# Autodesk Inventor assembly: Hexapod
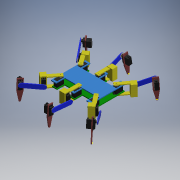
[picture p0: Inventor's stored thumbnail of the model, 180x180]
Saved by Autodesk Inventor 2017 (Build 210142000, 142)
## iProperties
Part Number: Hexapod
Document SubType Name: Assembly
Designer: alex-
Author: alex-
## Documents named in this file (7)
- D:\Alexander Miller\Documents\Git\Hexapod\3DParts\Hexapod.iam
- D:\Alexander Miller\Documents\Git\Hexapod\3DParts\Body_bottom.ipt
- D:\Alexander Miller\Documents\Git\Hexapod\3DParts\Serov_with_arm.iam
- D:\Alexander Miller\Documents\Git\Hexapod\3DParts\Body_top.ipt
- D:\Alexander Miller\Documents\Git\Hexapod\3DParts\Upper_leg.ipt
- D:\Alexander Miller\Documents\Git\Hexapod\3DParts\Middle_leg.ipt
- D:\Alexander Miller\Documents\Git\Hexapod\3DParts\Lower_leg.ipt
## Components (38 placed, 6 different names)
1. Body_bottom:1 — Rigid:1, Rigid:2, Rigid:3, Rigid:4, Rigid:5, Rigid:6
2. Serov_with_arm:1 [sub-assembly] — Rigid:1, Rigid:7, Rigid:40
3. Serov_with_arm:2 [sub-assembly] — Rigid:2, Rigid:41
4. Serov_with_arm:3 [sub-assembly] — Rigid:4, Rigid:42
5. Serov_with_arm:4 [sub-assembly] — Rigid:6, Rigid:43
6. Serov_with_arm:5 [sub-assembly] — Rigid:3, Rigid:39
7. Serov_with_arm:6 [sub-assembly] — Rigid:5, Rigid:38
8. Body_top:1 — Rigid:7
9. Upper_leg:1 — Rigid:8, Rigid:38
10. Upper_leg:2 — Rigid:15, Rigid:39
11. Upper_leg:3 — Rigid:16, Rigid:40
12. Upper_leg:4 — Rigid:19, Rigid:41
13. Upper_leg:5 — Rigid:18, Rigid:42
14. Upper_leg:6 — Rigid:17, Rigid:43
15. Serov_with_arm:7 [sub-assembly] — Rigid:8, Rigid:20
16. Serov_with_arm:8 [sub-assembly] — Rigid:17, Rigid:22
17. Serov_with_arm:9 [sub-assembly] — Rigid:19, Rigid:25
18. Serov_with_arm:10 [sub-assembly] — Rigid:16, Rigid:23
19. Serov_with_arm:11 [sub-assembly] — Rigid:18, Rigid:24
20. Serov_with_arm:12 [sub-assembly] — Rigid:15, Rigid:21
21. Middle_leg:1 — Rigid:20, Rigid:27
22. Middle_leg:2 — Rigid:22, Rigid:35
23. Middle_leg:3 — Rigid:25, Rigid:37
24. Middle_leg:4 — Rigid:24, Rigid:36
25. Middle_leg:5 — Rigid:23, Rigid:33
26. Middle_leg:6 — Rigid:21, Rigid:34
27. Serov_with_arm:13 [sub-assembly] — Rigid:26, Rigid:27
28. Serov_with_arm:14 [sub-assembly] — Rigid:28, Rigid:36
29. Serov_with_arm:15 [sub-assembly] — Rigid:30, Rigid:37
30. Serov_with_arm:16 [sub-assembly] — Rigid:32, Rigid:34
31. Serov_with_arm:17 [sub-assembly] — Rigid:31, Rigid:35
32. Serov_with_arm:18 [sub-assembly] — Rigid:29, Rigid:33
33. Lower_leg:1 — Rigid:26
34. Lower_leg:2 — Rigid:28
35. Lower_leg:3 — Rigid:29
36. Lower_leg:4 — Rigid:30
37. Lower_leg:5 — Rigid:31
38. Lower_leg:6 — Rigid:32
## Relationships (37: WeldJoint 37)
- Rigid:1 [WeldJoint]: Body_bottom:1 ↔ Serov_with_arm:1
- Rigid:2 [WeldJoint]: Body_bottom:1 ↔ Serov_with_arm:2
- Rigid:3 [WeldJoint]: Body_bottom:1 ↔ Serov_with_arm:5
- Rigid:4 [WeldJoint]: Body_bottom:1 ↔ Serov_with_arm:3
- Rigid:5 [WeldJoint]: Body_bottom:1 ↔ Serov_with_arm:6
- Rigid:6 [WeldJoint]: Body_bottom:1 ↔ Serov_with_arm:4
- Rigid:7 [WeldJoint]: Serov_with_arm:1 ↔ Body_top:1
- Rigid:8 [WeldJoint]: Upper_leg:1 ↔ Serov_with_arm:7
- Rigid:15 [WeldJoint]: Upper_leg:2 ↔ Serov_with_arm:12
- Rigid:16 [WeldJoint]: Upper_leg:3 ↔ Serov_with_arm:10
- Rigid:17 [WeldJoint]: Upper_leg:6 ↔ Serov_with_arm:8
- Rigid:18 [WeldJoint]: Upper_leg:5 ↔ Serov_with_arm:11
- Rigid:19 [WeldJoint]: Upper_leg:4 ↔ Serov_with_arm:9
- Rigid:20 [WeldJoint]: Serov_with_arm:7 ↔ Middle_leg:1
- Rigid:21 [WeldJoint]: Serov_with_arm:12 ↔ Middle_leg:6
- Rigid:23 [WeldJoint]: Serov_with_arm:10 ↔ Middle_leg:5
- Rigid:22 [WeldJoint]: Serov_with_arm:8 ↔ Middle_leg:2
- Rigid:24 [WeldJoint]: Serov_with_arm:11 ↔ Middle_leg:4
- Rigid:25 [WeldJoint]: Serov_with_arm:9 ↔ Middle_leg:3
- Rigid:26 [WeldJoint]: Serov_with_arm:13 ↔ Lower_leg:1
- Rigid:27 [WeldJoint]: Middle_leg:1 ↔ Serov_with_arm:13
- Rigid:28 [WeldJoint]: Serov_with_arm:14 ↔ Lower_leg:2
- Rigid:29 [WeldJoint]: Serov_with_arm:18 ↔ Lower_leg:3
- Rigid:30 [WeldJoint]: Serov_with_arm:15 ↔ Lower_leg:4
- Rigid:31 [WeldJoint]: Serov_with_arm:17 ↔ Lower_leg:5
- Rigid:32 [WeldJoint]: Serov_with_arm:16 ↔ Lower_leg:6
- Rigid:34 [WeldJoint]: Middle_leg:6 ↔ Serov_with_arm:16
- Rigid:33 [WeldJoint]: Middle_leg:5 ↔ Serov_with_arm:18
- Rigid:35 [WeldJoint]: Middle_leg:2 ↔ Serov_with_arm:17
- Rigid:36 [WeldJoint]: Middle_leg:4 ↔ Serov_with_arm:14
- Rigid:37 [WeldJoint]: Middle_leg:3 ↔ Serov_with_arm:15
- Rigid:38 [WeldJoint]: Serov_with_arm:6 ↔ Upper_leg:1
- Rigid:39 [WeldJoint]: Serov_with_arm:5 ↔ Upper_leg:2
- Rigid:40 [WeldJoint]: Serov_with_arm:1 ↔ Upper_leg:3
- Rigid:41 [WeldJoint]: Serov_with_arm:2 ↔ Upper_leg:4
- Rigid:42 [WeldJoint]: Serov_with_arm:3 ↔ Upper_leg:5
- Rigid:43 [WeldJoint]: Serov_with_arm:4 ↔ Upper_leg:6
